# Autodesk Inventor assembly: EjeconIman
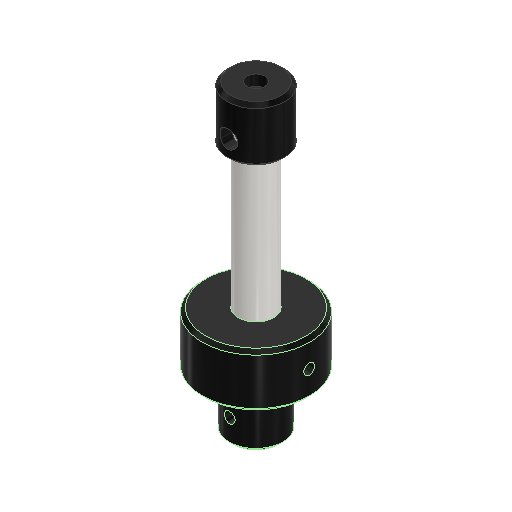
[picture p0: Inventor's stored thumbnail of the model, 512x512]
Saved by Autodesk Inventor 2025 (Build 290162000, 162)
## iProperties
Created: 2026-02-06
Part Number: EjeconIman
Document SubType Name: Assembly
Designer: HP
Author: HP
## Documents named in this file (4)
- C:\Users\HP\Desktop\TESIS 2\TFC2_20212123_MHinojosa\TFC2-20212123-HW\CAD\EjeconIman.iam
- C:\Users\HP\Desktop\TESIS 2\TFC2_20212123_MHinojosa\TFC2-20212123-HW\CAD\EJE.ipt
- C:\Users\HP\Desktop\TESIS 2\TFC2_20212123_MHinojosa\TFC2-20212123-HW\CAD\Acople_EJE.ipt
- C:\Users\HP\Desktop\TESIS 2\TFC2_20212123_MHinojosa\TFC2-20212123-HW\CAD\acople_iman.ipt
## Components (3 placed, 3 different names)
1. EJE:1 — Coincidencia:1, Coincidencia:2, Coincidencia:3, Coincidencia:4
2. Acople_EJE:1 — Coincidencia:1, Coincidencia:2
3. acople_iman:1 — Coincidencia:3, Coincidencia:4
## Relationships (4: Mate 4)
- Coincidencia:1 [Mate]: EJE:1 ↔ Acople_EJE:1
- Coincidencia:2 [Mate]: EJE:1 ↔ Acople_EJE:1
- Coincidencia:3 [Mate]: EJE:1 ↔ acople_iman:1
- Coincidencia:4 [Mate]: EJE:1 ↔ acople_iman:1
